# Autodesk Inventor assembly: Trunk
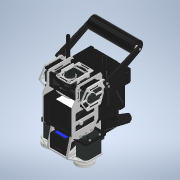
[picture p0: Inventor's stored thumbnail of the model, 180x180]
Saved by Autodesk Inventor 2020.4 (Build 244396000, 396)
## iProperties
Created: 2021-09-10
Part Number: Trunk
Document SubType Name: Assembly
Designer: Masato
Mass: 1534.62 g
Surface Area: 5672.23 cm^2
Volume: 933.606 cm^3
Density: 1.64375 g/cm^3
Author: Masato
## Documents named in this file (35)
- C:\Users\Masato\Documents\Inventor\CIT Brains_Inventor\OpenPlatform_ver3_0\UpperBody\Trunk\Trunk.iam
- C:\Users\Masato\Documents\Inventor\CIT Brains_Inventor\OpenPlatform_ver3_0\UpperBody\Trunk\Trunk_horizontal_frame_01.ipt
- C:\Users\Masato\Documents\Inventor\CIT Brains_Inventor\OpenPlatform_ver3_0\UpperBody\Trunk\Trunk_horizontal_frame_02.ipt
- C:\Users\Masato\Documents\Inventor\CIT Brains_Inventor\OpenPlatform_ver3_0\UpperBody\Trunk\Trunk_horizontal_frame_03.ipt
- C:\Users\Masato\Documents\Inventor\CIT Brains_Inventor\OpenPlatform_ver3_0\UpperBody\Trunk\Trunk_horizontal_frame_04.ipt
- C:\Users\Masato\Documents\Inventor\CIT Brains_Inventor\OpenPlatform_ver3_0\UpperBody\Trunk\Trunk_horizontal_frame_05.ipt
- C:\Users\Masato\Documents\Inventor\CIT Brains_Inventor\OpenPlatform_ver3_0\UpperBody\Trunk\Trunk_vertical_frame_02.ipt
- C:\Users\Masato\Documents\Inventor\CIT Brains_Inventor\OpenPlatform_ver3_0\UpperBody\Trunk\Trunk_vertical_frame_03.ipt
- C:\Users\Masato\Documents\Inventor\CIT Brains_Inventor\OpenPlatform_ver3_0\UpperBody\Trunk\Trunk_vertical_frame_04.ipt
- C:\Users\Masato\Documents\Inventor\CIT Brains_Inventor\OpenPlatform_ver3_0\UpperBody\Trunk\Trunk_vertical_frame_05.ipt
- C:\Users\Masato\Documents\Inventor\CIT Brains_Inventor\OpenPlatform_ver3_0\UpperBody\Trunk\Trunk_vertical_frame_06.ipt
- C:\Users\Masato\Documents\Inventor\CIT Brains_Inventor\OpenPlatform_ver3_0\Ready_Made\B3M11xx.ipt
- C:\Users\Masato\Documents\Inventor\CIT Brains_Inventor\OpenPlatform_ver3_0\Ready_Made\S3-07-3W.ipt
- C:\Users\Masato\Documents\Inventor\CIT Brains_Inventor\OpenPlatform_ver3_0\Ready_Made\ASU-375H.ipt
- C:\Users\Masato\Documents\Inventor\CIT Brains_Inventor\OpenPlatform_ver3_0\UpperBody\Trunk\RearBumper.ipt
- C:\Users\Masato\Documents\Inventor\CIT Brains_Inventor\OpenPlatform_ver3_0\UpperBody\Trunk\RearBumper_MIR.ipt
- C:\Users\Masato\Documents\Inventor\CIT Brains_Inventor\OpenPlatform_ver3_0\Ready_Made\MSU-306-03.ipt
- C:\Users\Masato\Documents\Inventor\CIT Brains_Inventor\OpenPlatform_ver3_0\Ready_Made\SLSBF7-130-M3-N3.ipt
- C:\Users\Masato\Documents\Inventor\CIT Brains_Inventor\OpenPlatform_ver3_0\Ready_Made\B3M10xx.ipt
- C:\Users\Masato\Documents\Inventor\CIT Brains_Inventor\OpenPlatform_ver3_0\Ready_Made\SGB-100.ipt
- C:\Users\Masato\Documents\Inventor\CIT Brains_Inventor\OpenPlatform_ver3_0\UpperBody\Cockpit\Cockpit.iam
- C:\Users\Masato\Documents\Inventor\CIT Brains_Inventor\OpenPlatform_ver3_0\UpperBody\Trunk\Trunk_vertical_frame_04_MIR.ipt
- C:\Users\Masato\Documents\Inventor\CIT Brains_Inventor\OpenPlatform_ver3_0\UpperBody\Trunk\Trunk_vertical_frame_01.ipt
- C:\Users\Masato\Documents\Inventor\CIT Brains_Inventor\OpenPlatform_ver3_0\UpperBody\Trunk\Trunk_vertical_frame_01_MIR.ipt
- C:\Users\Masato\Documents\Inventor\CIT Brains_Inventor\OpenPlatform_ver3_0\Ready_Made\Screw\SPNFL-BRN-M3-6.ipt
- C:\Users\Masato\Documents\Inventor\CIT Brains_Inventor\OpenPlatform_ver3_0\Ready_Made\Screw\M2_6-15.ipt
- C:\Users\Masato\Documents\Inventor\CIT Brains_Inventor\OpenPlatform_ver3_0\Ready_Made\Screw\M3-8.ipt
- C:\Users\Masato\Documents\Inventor\CIT Brains_Inventor\OpenPlatform_ver3_0\Ready_Made\Screw\M3-6.ipt
- C:\Users\Masato\Documents\Inventor\CIT Brains_Inventor\OpenPlatform_ver3_0\Ready_Made\Screw\M2_6-20.ipt
- C:\Users\Masato\Documents\Inventor\CIT Brains_Inventor\OpenPlatform_ver3_0\Thrust\Thrust_spacer_01.ipt
- C:\Users\Masato\Documents\Inventor\CIT Brains_Inventor\OpenPlatform_ver3_0\Ready_Made\83W-21.ipt
- C:\Users\Masato\Documents\Inventor\CIT Brains_Inventor\OpenPlatform_ver3_0\Ready_Made\CRBTF105AT.ipt
- C:\Users\Masato\Documents\Inventor\CIT Brains_Inventor\OpenPlatform_ver3_0\LowerBody\Leg_joit\Leg_joint_cross_bearing_frame.ipt
- C:\Users\Masato\Documents\Inventor\CIT Brains_Inventor\OpenPlatform_ver3_0\Ready_Made\Screw\M2_6-6.ipt
- C:\Users\Masato\Documents\Inventor\CIT Brains_Inventor\OpenPlatform_ver3_0\Ready_Made\Screw\No4_40-3-16.ipt
## Components (119 placed, 34 different names)
1. Trunk_horizontal_frame_01:1 — メイト:1, フラッシュ:14, 挿入:1, 挿入:2, 挿入:3, 挿入:4, 挿入:5, 挿入:6, 挿入:7, 挿入:8, 挿入:196, 挿入:197, 挿入:228, 挿入:233, 挿入:234, 挿入:237, 挿入:238, 挿入:241, 挿入:242, 挿入:243, 挿入:244, 挿入:273, 挿入:274, 挿入:275, 挿入:276
2. Trunk_horizontal_frame_02:1 — 挿入:9, 挿入:10, 挿入:11, 挿入:12, 挿入:269, 挿入:270, 挿入:271, 挿入:272
3. Trunk_horizontal_frame_03:1 — 挿入:172, 挿入:173, 挿入:174, 挿入:175, 挿入:176, 挿入:177, 挿入:178, 挿入:179, 挿入:255, 挿入:256, 挿入:259, 挿入:260, 挿入:261, 挿入:262
4. Trunk_horizontal_frame_03:2 — 挿入:180, 挿入:181, 挿入:182, 挿入:183, 挿入:184, 挿入:185, 挿入:186, 挿入:187, 挿入:257, 挿入:258
5. Trunk_horizontal_frame_04:1 — 挿入:115, 挿入:116, 挿入:117, 挿入:118, 挿入:172, 挿入:173, 挿入:181, 挿入:182
6. Trunk_horizontal_frame_04:2 — 挿入:154, 挿入:155, 挿入:156, 挿入:157, 挿入:174, 挿入:175, 挿入:185, 挿入:187
7. Trunk_horizontal_frame_05:1 — 挿入:111, 挿入:112, 挿入:126, 挿入:127
8. Trunk_horizontal_frame_05:2 — 挿入:162, 挿入:163, 挿入:164, 挿入:165
9. Trunk_horizontal_frame_05:3 — 挿入:229, 挿入:230, 挿入:231, 挿入:232
10. Trunk_horizontal_frame_05:4 — 挿入:166, 挿入:167, 挿入:168, 挿入:169
11. Trunk_vertical_frame_01:1 — 挿入:196, 挿入:197, 角度:35, 角度:36, 挿入:200, 挿入:201, 挿入:206, 挿入:207
12. Trunk_vertical_frame_01_MIR:1 — 角度:37, 角度:38, 挿入:202, 挿入:203, 挿入:204, 挿入:205, メイト:23, メイト:24, メイト:25, 挿入:228
13. Trunk_vertical_frame_02:1 — フラッシュ:16, メイト:17, フラッシュ:18, フラッシュ:20, フラッシュ:21, メイト:22
14. Trunk_vertical_frame_02:2 — フラッシュ:16, メイト:17, フラッシュ:18, メイト:19
15. Trunk_vertical_frame_02:3 — フラッシュ:15, メイト:18, フラッシュ:17, フラッシュ:19, フラッシュ:20, フラッシュ:21, メイト:21, メイト:20
16. Trunk_vertical_frame_02:4 — フラッシュ:15, メイト:18, フラッシュ:17, メイト:25
17. Trunk_vertical_frame_03:1 — 挿入:101, 挿入:102, 挿入:103, 挿入:111, 挿入:112, 挿入:115, 挿入:116, 挿入:156, 挿入:157, 挿入:164, 挿入:165, フラッシュ:19, メイト:21, 挿入:208, 挿入:226, 挿入:245, 挿入:246, 挿入:247, 挿入:251, 挿入:252
18. Trunk_vertical_frame_03:2 — 挿入:104, 挿入:105, 挿入:106, 挿入:117, 挿入:118, 挿入:154, 挿入:155, 挿入:168, 挿入:169, メイト:22, 挿入:227, 挿入:229, 挿入:230, 挿入:248, 挿入:249, 挿入:250, 挿入:253, 挿入:254
19. Trunk_vertical_frame_04:1 — 挿入:142, 挿入:143, 挿入:144, 挿入:145, 角度:31, 角度:32, 挿入:150, 挿入:151, 挿入:166, 挿入:167, 挿入:231, 挿入:232
20. Trunk_vertical_frame_04_MIR:1 — 挿入:124, 挿入:125, 挿入:126, 挿入:127, 挿入:128, 挿入:129, 挿入:136, 挿入:137, 角度:33, 角度:34, 挿入:152, 挿入:153, 挿入:162, 挿入:163
21. Trunk_vertical_frame_05:1 — 角度:17, 角度:18, 挿入:75, 挿入:76, 角度:21, 挿入:79, メイト:16, 挿入:263, 挿入:264, 挿入:267
22. Trunk_vertical_frame_05:2 — 角度:19, 挿入:77, 挿入:78, 角度:20, 角度:22, 挿入:80, 挿入:265, 挿入:266, 挿入:268
23. Trunk_vertical_frame_06:1 — 挿入:192, 挿入:193, 挿入:194, 挿入:195
24. Trunk_vertical_frame_06:2 — 挿入:188, 挿入:189, 挿入:190, 挿入:191
25. RearBumper:1 — 挿入:204, 挿入:205
26. RearBumper_MIR:1 — 挿入:206, 挿入:207
27. B3M11xx:1 — 挿入:1, 挿入:2, 挿入:3, 挿入:4, 挿入:11, 挿入:12, 角度:39, 挿入:281, 挿入:283, 挿入:285
28. B3M11xx:2 — 挿入:5, 挿入:6, 挿入:7, 挿入:8, 挿入:9, 挿入:10, 挿入:282, 挿入:284, 挿入:286
29. B3M11xx:3 — 挿入:176, 挿入:177, 挿入:178, 挿入:179, 挿入:180, 挿入:183, 挿入:184, 挿入:186
30. B3M10xx:4 — 挿入:124, 挿入:125, 挿入:128, 挿入:129, 挿入:188, 挿入:189, 挿入:190, 挿入:191
31. B3M10xx:5 — 挿入:142, 挿入:143, 挿入:144, 挿入:145, 挿入:192, 挿入:193, 挿入:194, 挿入:195
32. S3-07-3W:1 — 角度:37, 挿入:202
33. S3-07-3W:2 — 角度:38, 挿入:203
34. S3-07-3W:3 — 角度:36, 挿入:201
35. S3-07-3W:4 — 角度:35, 挿入:200
36. S3-07-3W:5 — 角度:33, 挿入:152
37. S3-07-3W:6 — 角度:34, 挿入:153
38. S3-07-3W:7 — 角度:31, 挿入:150
39. S3-07-3W:8 — 角度:32, 挿入:151
40. ASU-375H:1 — フラッシュ:9, フラッシュ:10, フラッシュ:11, フラッシュ:12, 挿入:101, 挿入:104, メイト:19, メイト:20, メイト:23, メイト:24
41. ASU-375H:2 — フラッシュ:9, フラッシュ:11, 挿入:102, 挿入:105
42. ASU-375H:3 — フラッシュ:10, フラッシュ:12, 挿入:103, 挿入:106
43. MSU-306-03:5 — 角度:17, 挿入:75, 挿入:136
44. MSU-306-03:6 — 角度:18, 挿入:76, 挿入:137
45. MSU-306-03:11 — 角度:19, 挿入:77
46. MSU-306-03:12 — 挿入:78, 角度:20
47. SLSBF7-130-M3-N3:1 — 角度:21, 角度:22, 挿入:79, 挿入:80, メイト:15
48. SGB-100:1 — メイト:15, メイト:16
49. Cockpit:1 [sub-assembly] — 挿入:208, 角度:39
50. SPNFL-BRN-M3-6:1 — 挿入:226
51. SPNFL-BRN-M3-6:2 — 挿入:227
52. M2_6-15:1 — 挿入:233
53. M2_6-15:2 — 挿入:234
54. M2_6-15:5 — 挿入:237
55. M2_6-15:6 — 挿入:238
56. M3-8:1 — 挿入:241
57. M3-8:2 — 挿入:242
58. M3-8:3 — 挿入:243
59. M3-8:4 — 挿入:244
60. M3-8:5 — 挿入:245
61. M3-8:6 — 挿入:246
62. M3-8:7 — 挿入:247
63. M3-8:8 — 挿入:248
64. M3-8:9 — 挿入:249
65. M3-8:10 — 挿入:250
66. M3-6:1 — 挿入:251
67. M3-6:2 — 挿入:252
68. M3-6:3 — 挿入:254
69. M3-6:4 — 挿入:253
70. M3-6:5 — 挿入:256
71. M3-6:6 — 挿入:255
72. M3-6:7 — 挿入:258
73. M3-6:8 — 挿入:257
74. M2_6-15:9 — 挿入:259
75. M2_6-15:10 — 挿入:260
76. M2_6-15:11 — 挿入:261
77. M2_6-15:12 — 挿入:262
78. M3-6:9 — 挿入:263
79. M3-6:10 — 挿入:264
80. M3-6:11 — 挿入:266
81. M3-6:12 — 挿入:265
82. M3-8:11 — 挿入:267
83. M3-8:12 — 挿入:268
84. M2_6-20:1 — 挿入:269
85. M2_6-20:2 — 挿入:270
86. M2_6-20:3 — 挿入:272
87. M2_6-20:4 — 挿入:271
88. Thrust_spacer_01:1 — 挿入:275, 挿入:276, 挿入:279, 挿入:280
89. Thrust_spacer_01:2 — 挿入:273, 挿入:274, 挿入:277, 挿入:278
90. M2_6-20:5 — 挿入:277
91. M2_6-20:6 — 挿入:278
92. M2_6-20:7 — 挿入:279
93. M2_6-20:8 — 挿入:280
94. 83W-21:1 — 挿入:281
95. 83W-21:2 — 挿入:282
96. CRBTF105AT:1 — 挿入:296, 挿入:297, 挿入:299, 挿入:300, 挿入:301, 挿入:302, 挿入:303, 挿入:304
97. CRBTF105AT:2 — 挿入:295, 挿入:298, 挿入:305, 挿入:306, 挿入:307, 挿入:308, 挿入:309, 挿入:310
98. Leg_joint_cross_bearing_frame:1 — 挿入:283, 挿入:285, 挿入:287, 挿入:288, 挿入:289, 挿入:290, 挿入:296, 挿入:297
99. Leg_joint_cross_bearing_frame:2 — 挿入:284, 挿入:286, 挿入:291, 挿入:292, 挿入:293, 挿入:294, 挿入:295, 挿入:298
100. M2_6-6:1 — 挿入:287
101. M2_6-6:2 — 挿入:288
102. M2_6-6:3 — 挿入:289
103. M2_6-6:4 — 挿入:290
104. M2_6-6:5 — 挿入:291
105. M2_6-6:6 — 挿入:292
106. M2_6-6:7 — 挿入:293
107. M2_6-6:8 — 挿入:294
108. No4_40-3-16:1 — 挿入:299
109. No4_40-3-16:2 — 挿入:300
110. No4_40-3-16:3 — 挿入:301
111. No4_40-3-16:4 — 挿入:302
112. No4_40-3-16:5 — 挿入:303
113. No4_40-3-16:6 — 挿入:304
114. No4_40-3-16:7 — 挿入:305
115. No4_40-3-16:8 — 挿入:306
116. No4_40-3-16:9 — 挿入:307
117. No4_40-3-16:10 — 挿入:308
118. No4_40-3-16:11 — 挿入:309
119. No4_40-3-16:12 — 挿入:310
## Relationships (213: Insert 174, Angle 15, Mate 12, Flush 12)
- メイト:1 [Mate]: Trunk_horizontal_frame_01:1
- フラッシュ:14 [Flush]: Trunk_horizontal_frame_01:1
- 挿入:1 [Insert]: Trunk_horizontal_frame_01:1 ↔ B3M11xx:1
- 挿入:2 [Insert]: Trunk_horizontal_frame_01:1 ↔ B3M11xx:1
- 挿入:3 [Insert]: Trunk_horizontal_frame_01:1 ↔ B3M11xx:1
- 挿入:4 [Insert]: Trunk_horizontal_frame_01:1 ↔ B3M11xx:1
- 挿入:5 [Insert]: Trunk_horizontal_frame_01:1 ↔ B3M11xx:2
- 挿入:6 [Insert]: Trunk_horizontal_frame_01:1 ↔ B3M11xx:2
- 挿入:7 [Insert]: Trunk_horizontal_frame_01:1 ↔ B3M11xx:2
- 挿入:8 [Insert]: Trunk_horizontal_frame_01:1 ↔ B3M11xx:2
- 挿入:9 [Insert]: Trunk_horizontal_frame_02:1 ↔ B3M11xx:2
- 挿入:10 [Insert]: Trunk_horizontal_frame_02:1 ↔ B3M11xx:2
- 挿入:11 [Insert]: Trunk_horizontal_frame_02:1 ↔ B3M11xx:1
- 挿入:12 [Insert]: Trunk_horizontal_frame_02:1 ↔ B3M11xx:1
- フラッシュ:9 [Flush]: ASU-375H:1 ↔ ASU-375H:2
- フラッシュ:10 [Flush]: ASU-375H:1 ↔ ASU-375H:3
- フラッシュ:11 [Flush]: ASU-375H:1 ↔ ASU-375H:2
- フラッシュ:12 [Flush]: ASU-375H:1 ↔ ASU-375H:3
- 角度:17 [Angle] (0 deg): Trunk_vertical_frame_05:1 ↔ MSU-306-03:5
- 角度:18 [Angle] (0 deg): Trunk_vertical_frame_05:1 ↔ MSU-306-03:6
- 挿入:75 [Insert]: Trunk_vertical_frame_05:1 ↔ MSU-306-03:5
- 挿入:76 [Insert]: Trunk_vertical_frame_05:1 ↔ MSU-306-03:6
- 角度:19 [Angle] (0 deg): Trunk_vertical_frame_05:2 ↔ MSU-306-03:11
- 挿入:77 [Insert]: Trunk_vertical_frame_05:2 ↔ MSU-306-03:11
- 挿入:78 [Insert]: Trunk_vertical_frame_05:2 ↔ MSU-306-03:12
- 角度:20 [Angle] (0 deg): Trunk_vertical_frame_05:2 ↔ MSU-306-03:12
- 角度:21 [Angle] (0 deg): Trunk_vertical_frame_05:1 ↔ SLSBF7-130-M3-N3:1
- 角度:22 [Angle] (0 deg): Trunk_vertical_frame_05:2 ↔ SLSBF7-130-M3-N3:1
- 挿入:79 [Insert]: Trunk_vertical_frame_05:1 ↔ SLSBF7-130-M3-N3:1
- 挿入:80 [Insert]: Trunk_vertical_frame_05:2 ↔ SLSBF7-130-M3-N3:1
- メイト:15 [Mate]: SLSBF7-130-M3-N3:1 ↔ SGB-100:1
- メイト:16 [Mate] (2.5 mm): Trunk_vertical_frame_05:1 ↔ SGB-100:1
- 挿入:101 [Insert]: Trunk_vertical_frame_03:1 ↔ ASU-375H:1
- 挿入:102 [Insert]: Trunk_vertical_frame_03:1 ↔ ASU-375H:2
- 挿入:103 [Insert]: Trunk_vertical_frame_03:1 ↔ ASU-375H:3
- 挿入:104 [Insert]: Trunk_vertical_frame_03:2 ↔ ASU-375H:1
- 挿入:105 [Insert]: Trunk_vertical_frame_03:2 ↔ ASU-375H:2
- 挿入:106 [Insert]: Trunk_vertical_frame_03:2 ↔ ASU-375H:3
- 挿入:111 [Insert]: Trunk_horizontal_frame_05:1 ↔ Trunk_vertical_frame_03:1
- 挿入:112 [Insert]: Trunk_horizontal_frame_05:1 ↔ Trunk_vertical_frame_03:1
- 挿入:115 [Insert]: Trunk_horizontal_frame_04:1 ↔ Trunk_vertical_frame_03:1
- 挿入:116 [Insert]: Trunk_horizontal_frame_04:1 ↔ Trunk_vertical_frame_03:1
- 挿入:117 [Insert]: Trunk_horizontal_frame_04:1 ↔ Trunk_vertical_frame_03:2
- 挿入:118 [Insert]: Trunk_horizontal_frame_04:1 ↔ Trunk_vertical_frame_03:2
- 挿入:124 [Insert]: Trunk_vertical_frame_04_MIR:1 ↔ B3M10xx:4
- 挿入:125 [Insert]: Trunk_vertical_frame_04_MIR:1 ↔ B3M10xx:4
- 挿入:126 [Insert]: Trunk_horizontal_frame_05:1 ↔ Trunk_vertical_frame_04_MIR:1
- 挿入:127 [Insert]: Trunk_horizontal_frame_05:1 ↔ Trunk_vertical_frame_04_MIR:1
- 挿入:128 [Insert]: Trunk_vertical_frame_04_MIR:1 ↔ B3M10xx:4
- 挿入:129 [Insert]: Trunk_vertical_frame_04_MIR:1 ↔ B3M10xx:4
- 挿入:136 [Insert]: Trunk_vertical_frame_04_MIR:1 ↔ MSU-306-03:5
- 挿入:137 [Insert]: Trunk_vertical_frame_04_MIR:1 ↔ MSU-306-03:6
- 挿入:142 [Insert]: Trunk_vertical_frame_04:1 ↔ B3M10xx:5
- 挿入:143 [Insert]: Trunk_vertical_frame_04:1 ↔ B3M10xx:5
- 挿入:144 [Insert]: Trunk_vertical_frame_04:1 ↔ B3M10xx:5
- 挿入:145 [Insert]: Trunk_vertical_frame_04:1 ↔ B3M10xx:5
- 角度:31 [Angle] (0 deg): Trunk_vertical_frame_04:1 ↔ S3-07-3W:7
- 角度:32 [Angle] (0 deg): Trunk_vertical_frame_04:1 ↔ S3-07-3W:8
- 挿入:150 [Insert]: Trunk_vertical_frame_04:1 ↔ S3-07-3W:7
- 挿入:151 [Insert]: Trunk_vertical_frame_04:1 ↔ S3-07-3W:8
- 角度:33 [Angle] (0 deg): Trunk_vertical_frame_04_MIR:1 ↔ S3-07-3W:5
- 角度:34 [Angle] (0 deg): Trunk_vertical_frame_04_MIR:1 ↔ S3-07-3W:6
- 挿入:152 [Insert]: Trunk_vertical_frame_04_MIR:1 ↔ S3-07-3W:5
- 挿入:153 [Insert]: Trunk_vertical_frame_04_MIR:1 ↔ S3-07-3W:6
- 挿入:154 [Insert]: Trunk_horizontal_frame_04:2 ↔ Trunk_vertical_frame_03:2
- 挿入:155 [Insert]: Trunk_horizontal_frame_04:2 ↔ Trunk_vertical_frame_03:2
- 挿入:156 [Insert]: Trunk_horizontal_frame_04:2 ↔ Trunk_vertical_frame_03:1
- 挿入:157 [Insert]: Trunk_horizontal_frame_04:2 ↔ Trunk_vertical_frame_03:1
- 挿入:162 [Insert]: Trunk_horizontal_frame_05:2 ↔ Trunk_vertical_frame_04_MIR:1
- 挿入:163 [Insert]: Trunk_horizontal_frame_05:2 ↔ Trunk_vertical_frame_04_MIR:1
- 挿入:164 [Insert]: Trunk_horizontal_frame_05:2 ↔ Trunk_vertical_frame_03:1
- 挿入:165 [Insert]: Trunk_horizontal_frame_05:2 ↔ Trunk_vertical_frame_03:1
- 挿入:166 [Insert]: Trunk_horizontal_frame_05:4 ↔ Trunk_vertical_frame_04:1
- 挿入:167 [Insert]: Trunk_horizontal_frame_05:4 ↔ Trunk_vertical_frame_04:1
- 挿入:168 [Insert]: Trunk_horizontal_frame_05:4 ↔ Trunk_vertical_frame_03:2
- 挿入:169 [Insert]: Trunk_horizontal_frame_05:4 ↔ Trunk_vertical_frame_03:2
- 挿入:172 [Insert]: Trunk_horizontal_frame_03:1 ↔ Trunk_horizontal_frame_04:1
- 挿入:173 [Insert]: Trunk_horizontal_frame_03:1 ↔ Trunk_horizontal_frame_04:1
- 挿入:174 [Insert]: Trunk_horizontal_frame_03:1 ↔ Trunk_horizontal_frame_04:2
- 挿入:175 [Insert]: Trunk_horizontal_frame_03:1 ↔ Trunk_horizontal_frame_04:2
- 挿入:176 [Insert]: Trunk_horizontal_frame_03:1 ↔ B3M11xx:3
- 挿入:177 [Insert]: Trunk_horizontal_frame_03:1 ↔ B3M11xx:3
- 挿入:178 [Insert]: Trunk_horizontal_frame_03:1 ↔ B3M11xx:3
- 挿入:179 [Insert]: Trunk_horizontal_frame_03:1 ↔ B3M11xx:3
- 挿入:180 [Insert]: Trunk_horizontal_frame_03:2 ↔ B3M11xx:3
- 挿入:181 [Insert]: Trunk_horizontal_frame_03:2 ↔ Trunk_horizontal_frame_04:1
- 挿入:182 [Insert]: Trunk_horizontal_frame_03:2 ↔ Trunk_horizontal_frame_04:1
- 挿入:183 [Insert]: Trunk_horizontal_frame_03:2 ↔ B3M11xx:3
- 挿入:184 [Insert]: Trunk_horizontal_frame_03:2 ↔ B3M11xx:3
- 挿入:185 [Insert]: Trunk_horizontal_frame_03:2 ↔ Trunk_horizontal_frame_04:2
- 挿入:186 [Insert]: Trunk_horizontal_frame_03:2 ↔ B3M11xx:3
- 挿入:187 [Insert]: Trunk_horizontal_frame_03:2 ↔ Trunk_horizontal_frame_04:2
- 挿入:188 [Insert]: Trunk_vertical_frame_06:2 ↔ B3M10xx:4
- 挿入:189 [Insert]: Trunk_vertical_frame_06:2 ↔ B3M10xx:4
- 挿入:190 [Insert]: Trunk_vertical_frame_06:2 ↔ B3M10xx:4
- 挿入:191 [Insert]: Trunk_vertical_frame_06:2 ↔ B3M10xx:4
- 挿入:192 [Insert]: Trunk_vertical_frame_06:1 ↔ B3M10xx:5
- 挿入:193 [Insert]: Trunk_vertical_frame_06:1 ↔ B3M10xx:5
- 挿入:194 [Insert]: Trunk_vertical_frame_06:1 ↔ B3M10xx:5
- 挿入:195 [Insert]: Trunk_vertical_frame_06:1 ↔ B3M10xx:5
- フラッシュ:15 [Flush]: Trunk_vertical_frame_02:3 ↔ Trunk_vertical_frame_02:4
- フラッシュ:16 [Flush]: Trunk_vertical_frame_02:1 ↔ Trunk_vertical_frame_02:2
- メイト:17 [Mate]: Trunk_vertical_frame_02:1 ↔ Trunk_vertical_frame_02:2
- メイト:18 [Mate]: Trunk_vertical_frame_02:3 ↔ Trunk_vertical_frame_02:4
- フラッシュ:17 [Flush]: Trunk_vertical_frame_02:3 ↔ Trunk_vertical_frame_02:4
- フラッシュ:18 [Flush]: Trunk_vertical_frame_02:1 ↔ Trunk_vertical_frame_02:2
- フラッシュ:19 [Flush]: Trunk_vertical_frame_02:3 ↔ Trunk_vertical_frame_03:1
- フラッシュ:20 [Flush]: Trunk_vertical_frame_02:1 ↔ Trunk_vertical_frame_02:3
- メイト:19 [Mate] (0.01 mm): Trunk_vertical_frame_02:2 ↔ ASU-375H:1
- メイト:20 [Mate] (0.01 mm): Trunk_vertical_frame_02:3 ↔ ASU-375H:1
- フラッシュ:21 [Flush]: Trunk_vertical_frame_02:1 ↔ Trunk_vertical_frame_02:3
- メイト:21 [Mate]: Trunk_vertical_frame_02:3 ↔ Trunk_vertical_frame_03:1
- メイト:22 [Mate]: Trunk_vertical_frame_02:1 ↔ Trunk_vertical_frame_03:2
- 挿入:196 [Insert]: Trunk_horizontal_frame_01:1 ↔ Trunk_vertical_frame_01:1
- 挿入:197 [Insert]: Trunk_horizontal_frame_01:1 ↔ Trunk_vertical_frame_01:1
- 角度:35 [Angle] (0 deg): Trunk_vertical_frame_01:1 ↔ S3-07-3W:4
- 角度:36 [Angle] (0 deg): Trunk_vertical_frame_01:1 ↔ S3-07-3W:3
- 挿入:200 [Insert]: Trunk_vertical_frame_01:1 ↔ S3-07-3W:4
- 挿入:201 [Insert]: Trunk_vertical_frame_01:1 ↔ S3-07-3W:3
- 角度:37 [Angle] (0 deg): Trunk_vertical_frame_01_MIR:1 ↔ S3-07-3W:1
- 角度:38 [Angle] (0 deg): Trunk_vertical_frame_01_MIR:1 ↔ S3-07-3W:2
- 挿入:202 [Insert]: Trunk_vertical_frame_01_MIR:1 ↔ S3-07-3W:1
- 挿入:203 [Insert]: Trunk_vertical_frame_01_MIR:1 ↔ S3-07-3W:2
- 挿入:204 [Insert]: Trunk_vertical_frame_01_MIR:1 ↔ RearBumper:1
- 挿入:205 [Insert]: Trunk_vertical_frame_01_MIR:1 ↔ RearBumper:1
- 挿入:206 [Insert]: Trunk_vertical_frame_01:1 ↔ RearBumper_MIR:1
- 挿入:207 [Insert]: Trunk_vertical_frame_01:1 ↔ RearBumper_MIR:1
- メイト:23 [Mate] (0.01 mm): Trunk_vertical_frame_01_MIR:1 ↔ ASU-375H:1
- メイト:24 [Mate] (0.01 mm): Trunk_vertical_frame_01_MIR:1 ↔ ASU-375H:1
- メイト:25 [Mate]: Trunk_vertical_frame_01_MIR:1 ↔ Trunk_vertical_frame_02:4
- 挿入:208 [Insert] (0.25 mm): Trunk_vertical_frame_03:1 ↔ Cockpit:1
- 角度:39 [Angle] (0 deg): B3M11xx:1 ↔ Cockpit:1
- 挿入:226 [Insert]: Trunk_vertical_frame_03:1 ↔ SPNFL-BRN-M3-6:1
- 挿入:227 [Insert]: Trunk_vertical_frame_03:2 ↔ SPNFL-BRN-M3-6:2
- 挿入:228 [Insert]: Trunk_horizontal_frame_01:1 ↔ Trunk_vertical_frame_01_MIR:1
- 挿入:229 [Insert]: Trunk_horizontal_frame_05:3 ↔ Trunk_vertical_frame_03:2
- 挿入:230 [Insert]: Trunk_horizontal_frame_05:3 ↔ Trunk_vertical_frame_03:2
- 挿入:231 [Insert]: Trunk_horizontal_frame_05:3 ↔ Trunk_vertical_frame_04:1
- 挿入:232 [Insert]: Trunk_horizontal_frame_05:3 ↔ Trunk_vertical_frame_04:1
- 挿入:233 [Insert]: Trunk_horizontal_frame_01:1 ↔ M2_6-15:1
- 挿入:234 [Insert]: Trunk_horizontal_frame_01:1 ↔ M2_6-15:2
- 挿入:237 [Insert]: Trunk_horizontal_frame_01:1 ↔ M2_6-15:5
- 挿入:238 [Insert]: Trunk_horizontal_frame_01:1 ↔ M2_6-15:6
- 挿入:241 [Insert]: Trunk_horizontal_frame_01:1 ↔ M3-8:1
- 挿入:242 [Insert]: Trunk_horizontal_frame_01:1 ↔ M3-8:2
- 挿入:243 [Insert]: Trunk_horizontal_frame_01:1 ↔ M3-8:3
- 挿入:244 [Insert]: Trunk_horizontal_frame_01:1 ↔ M3-8:4
- 挿入:245 [Insert]: Trunk_vertical_frame_03:1 ↔ M3-8:5
- 挿入:246 [Insert]: Trunk_vertical_frame_03:1 ↔ M3-8:6
- 挿入:247 [Insert]: Trunk_vertical_frame_03:1 ↔ M3-8:7
- 挿入:248 [Insert]: Trunk_vertical_frame_03:2 ↔ M3-8:8
- 挿入:249 [Insert]: Trunk_vertical_frame_03:2 ↔ M3-8:9
- 挿入:250 [Insert]: Trunk_vertical_frame_03:2 ↔ M3-8:10
- 挿入:251 [Insert]: Trunk_vertical_frame_03:1 ↔ M3-6:1
- 挿入:252 [Insert]: Trunk_vertical_frame_03:1 ↔ M3-6:2
- 挿入:253 [Insert]: Trunk_vertical_frame_03:2 ↔ M3-6:4
- 挿入:254 [Insert]: Trunk_vertical_frame_03:2 ↔ M3-6:3
- 挿入:255 [Insert]: Trunk_horizontal_frame_03:1 ↔ M3-6:6
- 挿入:256 [Insert]: Trunk_horizontal_frame_03:1 ↔ M3-6:5
- 挿入:257 [Insert]: Trunk_horizontal_frame_03:2 ↔ M3-6:8
- 挿入:258 [Insert]: Trunk_horizontal_frame_03:2 ↔ M3-6:7
- 挿入:259 [Insert]: Trunk_horizontal_frame_03:1 ↔ M2_6-15:9
- 挿入:260 [Insert]: Trunk_horizontal_frame_03:1 ↔ M2_6-15:10
- 挿入:261 [Insert]: Trunk_horizontal_frame_03:1 ↔ M2_6-15:11
- 挿入:262 [Insert]: Trunk_horizontal_frame_03:1 ↔ M2_6-15:12
- 挿入:263 [Insert]: Trunk_vertical_frame_05:1 ↔ M3-6:9
- 挿入:264 [Insert]: Trunk_vertical_frame_05:1 ↔ M3-6:10
- 挿入:265 [Insert]: Trunk_vertical_frame_05:2 ↔ M3-6:12
- 挿入:266 [Insert]: Trunk_vertical_frame_05:2 ↔ M3-6:11
- 挿入:267 [Insert]: Trunk_vertical_frame_05:1 ↔ M3-8:11
- 挿入:268 [Insert]: Trunk_vertical_frame_05:2 ↔ M3-8:12
- 挿入:269 [Insert]: Trunk_horizontal_frame_02:1 ↔ M2_6-20:1
- 挿入:270 [Insert]: Trunk_horizontal_frame_02:1 ↔ M2_6-20:2
- 挿入:271 [Insert]: Trunk_horizontal_frame_02:1 ↔ M2_6-20:4
- 挿入:272 [Insert]: Trunk_horizontal_frame_02:1 ↔ M2_6-20:3
- 挿入:273 [Insert]: Trunk_horizontal_frame_01:1 ↔ Thrust_spacer_01:2
- 挿入:274 [Insert]: Trunk_horizontal_frame_01:1 ↔ Thrust_spacer_01:2
- 挿入:275 [Insert]: Trunk_horizontal_frame_01:1 ↔ Thrust_spacer_01:1
- 挿入:276 [Insert]: Trunk_horizontal_frame_01:1 ↔ Thrust_spacer_01:1
- 挿入:277 [Insert]: Thrust_spacer_01:2 ↔ M2_6-20:5
- 挿入:278 [Insert]: Thrust_spacer_01:2 ↔ M2_6-20:6
- 挿入:279 [Insert]: Thrust_spacer_01:1 ↔ M2_6-20:7
- 挿入:280 [Insert]: Thrust_spacer_01:1 ↔ M2_6-20:8
- 挿入:281 [Insert]: B3M11xx:1 ↔ 83W-21:1
- 挿入:282 [Insert]: B3M11xx:2 ↔ 83W-21:2
- 挿入:283 [Insert]: B3M11xx:1 ↔ Leg_joint_cross_bearing_frame:1
- 挿入:284 [Insert]: B3M11xx:2 ↔ Leg_joint_cross_bearing_frame:2
- 挿入:285 [Insert]: B3M11xx:1 ↔ Leg_joint_cross_bearing_frame:1
- 挿入:286 [Insert]: B3M11xx:2 ↔ Leg_joint_cross_bearing_frame:2
- 挿入:287 [Insert]: Leg_joint_cross_bearing_frame:1 ↔ M2_6-6:1
- 挿入:288 [Insert]: Leg_joint_cross_bearing_frame:1 ↔ M2_6-6:2
- 挿入:289 [Insert]: Leg_joint_cross_bearing_frame:1 ↔ M2_6-6:3
- 挿入:290 [Insert]: Leg_joint_cross_bearing_frame:1 ↔ M2_6-6:4
- 挿入:291 [Insert]: Leg_joint_cross_bearing_frame:2 ↔ M2_6-6:5
- 挿入:292 [Insert]: Leg_joint_cross_bearing_frame:2 ↔ M2_6-6:6
- 挿入:293 [Insert]: Leg_joint_cross_bearing_frame:2 ↔ M2_6-6:7
- 挿入:294 [Insert]: Leg_joint_cross_bearing_frame:2 ↔ M2_6-6:8
- 挿入:295 [Insert]: CRBTF105AT:2 ↔ Leg_joint_cross_bearing_frame:2
- 挿入:296 [Insert]: CRBTF105AT:1 ↔ Leg_joint_cross_bearing_frame:1
- 挿入:297 [Insert]: CRBTF105AT:1 ↔ Leg_joint_cross_bearing_frame:1
- 挿入:298 [Insert]: CRBTF105AT:2 ↔ Leg_joint_cross_bearing_frame:2
- 挿入:299 [Insert]: CRBTF105AT:1 ↔ No4_40-3-16:1
- 挿入:300 [Insert]: CRBTF105AT:1 ↔ No4_40-3-16:2
- 挿入:301 [Insert]: CRBTF105AT:1 ↔ No4_40-3-16:3
- 挿入:302 [Insert]: CRBTF105AT:1 ↔ No4_40-3-16:4
- 挿入:303 [Insert]: CRBTF105AT:1 ↔ No4_40-3-16:5
- 挿入:304 [Insert]: CRBTF105AT:1 ↔ No4_40-3-16:6
- 挿入:305 [Insert]: CRBTF105AT:2 ↔ No4_40-3-16:7
- 挿入:306 [Insert]: CRBTF105AT:2 ↔ No4_40-3-16:8
- 挿入:307 [Insert]: CRBTF105AT:2 ↔ No4_40-3-16:9
- 挿入:308 [Insert]: CRBTF105AT:2 ↔ No4_40-3-16:10
- 挿入:309 [Insert]: CRBTF105AT:2 ↔ No4_40-3-16:11
- 挿入:310 [Insert]: CRBTF105AT:2 ↔ No4_40-3-16:12
